# Autodesk Inventor assembly: demo
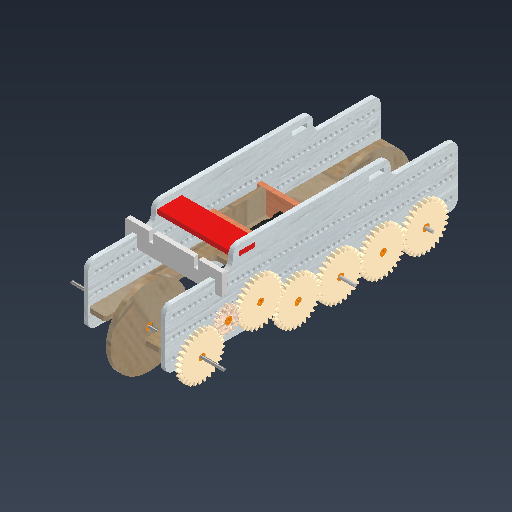
[picture p0: Inventor's stored thumbnail of the model, 512x512]
Saved by Autodesk Inventor 2025.3 (Build 293356000, 356)
## iProperties
Created: 2025-11-06
Part Number: demo
Document SubType Name: Assembly
Designer: 陳泓任
Mass: 93.4584 g
Surface Area: 978.247 cm^2
Volume: 113.725 cm^3
Density: 0.82179 g/cm^3
Author: 陳泓任
## Documents named in this file (19)
- C:\Users\Ou918\3D-model-temp\introduction to mechanical engineering(1)\version_7\demo.iam
- C:\Users\Ou918\3D-model-temp\introduction to mechanical engineering(1)\發條組合\發條組合.iam
- C:\Users\Ou918\3D-model-temp\introduction to mechanical engineering(1)\version_6\baffle_back_short.ipt
- C:\Users\Ou918\3D-model-temp\introduction to mechanical engineering(1)\version_6\baffle_front_short.ipt
- C:\Users\Ou918\3D-model-temp\introduction to mechanical engineering(1)\version_6\beam.ipt
- C:\Users\Ou918\3D-model-temp\introduction to mechanical engineering(1)\version_5\support_edited.ipt
- C:\Users\Ou918\3D-model-temp\introduction to mechanical engineering(1)\version_5\bolt.ipt
- C:\Users\Ou918\3D-model-temp\introduction to mechanical engineering(1)\sleeve.ipt
- C:\Users\Ou918\3D-model-temp\introduction to mechanical engineering(1)\big gear(with sleeve).iam
- C:\Users\Ou918\3D-model-temp\introduction to mechanical engineering(1)\51mm wheel(with sleeve).iam
- C:\Users\Ou918\3D-model-temp\introduction to mechanical engineering(1)\100mm rod.ipt
- C:\Users\Ou918\3D-model-temp\introduction to mechanical engineering(1)\80mm rod.ipt
- C:\Users\Ou918\3D-model-temp\introduction to mechanical engineering(1)\small gear(with sleeve).iam
- C:\Users\Ou918\3D-model-temp\introduction to mechanical engineering(1)\version_7\main_frame(short).ipt
- C:\Users\Ou918\3D-model-temp\introduction to mechanical engineering(1)\version_7\beam.ipt
- C:\Users\Ou918\3D-model-temp\introduction to mechanical engineering(1)\version_7\side_frame_revised.ipt
- C:\Users\Ou918\3D-model-temp\introduction to mechanical engineering(1)\middle gear.iam
- C:\Users\Ou918\3D-model-temp\introduction to mechanical engineering(1)\version_7\main_frame_long.ipt
- C:\Users\Ou918\3D-model-temp\introduction to mechanical engineering(1)\version_7\brackt.ipt
## Components (31 placed, 17 different names)
1. main_frame(short):1 — 貼合:48, 貼合:49, 貼合:50, 齊平:7, 貼合:51, 貼合:55, 角度:2, 齊平:8, 貼合:60, 貼合:61, 貼合:64, 貼合:65, 齊平:12
2. 發條組合:1 [sub-assembly] — 貼合:16, 貼合:31, 貼合:32, 齊平:7, 貼合:55, 貼合:68, 貼合:81
3. side_frame_revised:1 — 貼合:62, 齊平:9, 貼合:63, 貼合:64, 貼合:70, 貼合:71, 齊平:10, 貼合:73, 角度:3, 貼合:74, 貼合:75, 貼合:76, 貼合:77, 貼合:78, 貼合:83, 貼合:84, 貼合:85
4. side_frame_revised:2 — 貼合:65, 貼合:66, 貼合:67, 貼合:68, 貼合:72, 貼合:86, 貼合:87
5. baffle_back_short:1 — 貼合:20, 貼合:26, 貼合:53, 貼合:54, 貼合:56
6. baffle_front_short:1 — 貼合:16, 貼合:23, 貼合:25, 貼合:49, 貼合:51, 貼合:52
7. beam:2 — 貼合:62, 齊平:9, 貼合:63, 貼合:66, 貼合:67
8. support_edited:1 — 貼合:20, 貼合:23, 貼合:27, 貼合:29, 貼合:48, 貼合:50, 貼合:52, 貼合:53, 貼合:54
9. support_edited:2 — 貼合:25, 貼合:26, 貼合:28, 貼合:56, 貼合:79, 貼合:80
10. bolt:1 — 貼合:27, 貼合:28, 貼合:29
11. sleeve:1 — 貼合:31, 貼合:33, 貼合:71
12. big gear(with sleeve):1 [sub-assembly] — 貼合:32, 貼合:33, 齊平:2, 齊平:5, 貼合:82
13. big gear(with sleeve):2 [sub-assembly] — with_gear, 齊平:3, 齊平:6
14. 51mm wheel(with sleeve):1 [sub-assembly] — with_wheel
15. 51mm wheel(with sleeve):3 [sub-assembly] — 貼合:45
16. 100mm rod:1 — 貼合:38, 貼合:60, with_gear, with_wheel, 貼合:78
17. sleeve:2 — 貼合:38
18. big gear(with sleeve):3 [sub-assembly] — 齊平:1, 齊平:11, 貼合:77
19. big gear(with sleeve):5 [sub-assembly] — 齊平:4, 齊平:5
20. big gear(with sleeve):6 [sub-assembly] — 齊平:4, 貼合:43
21. 80mm rod:1 — 貼合:43, 貼合:45, 貼合:61, 貼合:70
22. big gear(with sleeve):4 [sub-assembly] — 齊平:1, 齊平:2, 齊平:3, 貼合:74
23. small gear(with sleeve):1 [sub-assembly] — 齊平:6, 貼合:76
24. beam:3 — 貼合:72, 齊平:10, 貼合:73
25. big gear(with sleeve):7 [sub-assembly] — 齊平:11, 貼合:75
26. middle gear:1 [sub-assembly] — 貼合:81, 齊平:13, 貼合:82
27. main_frame_long:1 — 齊平:12, 貼合:79, 貼合:80
28. middle gear:2 [sub-assembly] — 齊平:13, 齊平:14, 貼合:83
29. middle gear:3 [sub-assembly] — 齊平:14, 齊平:15, 貼合:84
30. middle gear:4 [sub-assembly] — 齊平:15, 貼合:85
31. brackt:1 — 貼合:86, 貼合:87
## Relationships (69: Mate 52, Flush 15, Angle 2)
- 貼合:16 [Mate]: 發條組合:1 ↔ baffle_front_short:1
- 貼合:20 [Mate]: baffle_back_short:1 ↔ support_edited:1
- 貼合:23 [Mate]: baffle_front_short:1 ↔ support_edited:1
- 貼合:25 [Mate]: baffle_front_short:1 ↔ support_edited:2
- 貼合:26 [Mate]: baffle_back_short:1 ↔ support_edited:2
- 貼合:27 [Mate]: support_edited:1 ↔ bolt:1
- 貼合:28 [Mate]: support_edited:2 ↔ bolt:1
- 貼合:29 [Mate]: support_edited:1 ↔ bolt:1
- 貼合:31 [Mate]: 發條組合:1 ↔ sleeve:1
- 貼合:32 [Mate]: 發條組合:1 ↔ big gear(with sleeve):1
- 貼合:33 [Mate]: sleeve:1 ↔ big gear(with sleeve):1
- 貼合:38 [Mate]: 100mm rod:1 ↔ sleeve:2
- 貼合:60 [Mate]: main_frame(short):1 ↔ 100mm rod:1
- with_gear [Mate]: big gear(with sleeve):2 ↔ 100mm rod:1
- with_wheel [Mate]: 51mm wheel(with sleeve):1 ↔ 100mm rod:1
- 齊平:1 [Flush]: big gear(with sleeve):3 ↔ big gear(with sleeve):4
- 齊平:2 [Flush]: big gear(with sleeve):1 ↔ big gear(with sleeve):4
- 齊平:3 [Flush]: big gear(with sleeve):2 ↔ big gear(with sleeve):4
- 齊平:4 [Flush]: big gear(with sleeve):5 ↔ big gear(with sleeve):6
- 齊平:5 [Flush]: big gear(with sleeve):1 ↔ big gear(with sleeve):5
- 貼合:43 [Mate]: big gear(with sleeve):6 ↔ 80mm rod:1
- 貼合:45 [Mate]: 51mm wheel(with sleeve):3 ↔ 80mm rod:1
- 齊平:6 [Flush]: big gear(with sleeve):2 ↔ small gear(with sleeve):1
- 貼合:48 [Mate]: main_frame(short):1 ↔ support_edited:1
- 貼合:49 [Mate]: main_frame(short):1 ↔ baffle_front_short:1
- 貼合:50 [Mate]: main_frame(short):1 ↔ support_edited:1
- 齊平:7 [Flush] (-6.75 mm): main_frame(short):1 ↔ 發條組合:1
- 貼合:51 [Mate]: main_frame(short):1 ↔ baffle_front_short:1
- 貼合:52 [Mate]: baffle_front_short:1 ↔ support_edited:1
- 貼合:53 [Mate]: baffle_back_short:1 ↔ support_edited:1
- 貼合:54 [Mate]: baffle_back_short:1 ↔ support_edited:1
- 貼合:55 [Mate]: main_frame(short):1 ↔ 發條組合:1
- 貼合:56 [Mate]: baffle_back_short:1 ↔ support_edited:2
- 角度:2 [Angle] (0 deg): main_frame(short):1
- 齊平:8 [Flush]: main_frame(short):1
- 貼合:61 [Mate]: main_frame(short):1 ↔ 80mm rod:1
- 貼合:62 [Mate]: side_frame_revised:1 ↔ beam:2
- 齊平:9 [Flush]: side_frame_revised:1 ↔ beam:2
- 貼合:63 [Mate]: side_frame_revised:1 ↔ beam:2
- 貼合:64 [Mate]: main_frame(short):1 ↔ side_frame_revised:1
- 貼合:65 [Mate]: main_frame(short):1 ↔ side_frame_revised:2
- 貼合:66 [Mate]: side_frame_revised:2 ↔ beam:2
- 貼合:67 [Mate]: side_frame_revised:2 ↔ beam:2
- 貼合:68 [Mate]: 發條組合:1 ↔ side_frame_revised:2
- 貼合:70 [Mate]: side_frame_revised:1 ↔ 80mm rod:1
- 貼合:71 [Mate] (3 mm): side_frame_revised:1 ↔ sleeve:1
- 貼合:72 [Mate]: side_frame_revised:2 ↔ beam:3
- 齊平:10 [Flush]: side_frame_revised:1 ↔ beam:3
- 貼合:73 [Mate]: side_frame_revised:1 ↔ beam:3
- 角度:3 [Angle] (0 deg): side_frame_revised:1
- 貼合:74 [Mate]: side_frame_revised:1 ↔ big gear(with sleeve):4
- 齊平:11 [Flush]: big gear(with sleeve):3 ↔ big gear(with sleeve):7
- 貼合:75 [Mate]: side_frame_revised:1 ↔ big gear(with sleeve):7
- 貼合:76 [Mate]: side_frame_revised:1 ↔ small gear(with sleeve):1
- 貼合:77 [Mate]: side_frame_revised:1 ↔ big gear(with sleeve):3
- 貼合:78 [Mate]: side_frame_revised:1 ↔ 100mm rod:1
- 齊平:12 [Flush]: main_frame(short):1 ↔ main_frame_long:1
- 貼合:79 [Mate]: support_edited:2 ↔ main_frame_long:1
- 貼合:80 [Mate]: support_edited:2 ↔ main_frame_long:1
- 貼合:81 [Mate]: 發條組合:1 ↔ middle gear:1
- 齊平:13 [Flush]: middle gear:1 ↔ middle gear:2
- 貼合:82 [Mate] (3 mm): big gear(with sleeve):1 ↔ middle gear:1
- 齊平:14 [Flush]: middle gear:2 ↔ middle gear:3
- 齊平:15 [Flush]: middle gear:3 ↔ middle gear:4
- 貼合:83 [Mate]: side_frame_revised:1 ↔ middle gear:2
- 貼合:84 [Mate]: side_frame_revised:1 ↔ middle gear:3
- 貼合:85 [Mate]: side_frame_revised:1 ↔ middle gear:4
- 貼合:86 [Mate]: side_frame_revised:2 ↔ brackt:1
- 貼合:87 [Mate]: side_frame_revised:2 ↔ brackt:1
